# Autodesk Inventor assembly: MOTOR ENSAMBLE
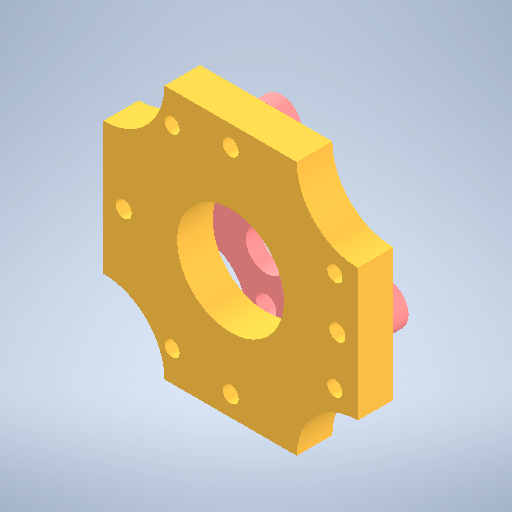
[picture p0: Inventor's stored thumbnail of the model, 512x512]
Saved by Autodesk Inventor 2025.3 (Build 293356030, 356C)
## iProperties
Created: 2025-07-11
Part Number: MOTOR ENSAMBLE
Document SubType Name: Assembly
Designer: jv
Author: jv
## Documents named in this file (3)
- C:\Users\jv\Downloads\MODELOS NUEVOS\MOTOR\MOTOR ENSAMBLE.iam
- C:\Users\jv\Downloads\MODELOS NUEVOS\MOTOR\CONECTOR DE ACOPLE A AVION.ipt
- C:\Users\jv\Downloads\MODELOS NUEVOS\MOTOR\ACOPLE.ipt
## Components (2 placed, 2 different names)
1. CONECTOR DE ACOPLE A AVION:1 — Mate:1
2. ACOPLE:1 — Mate:1
## Relationships (1: Mate 1)
- Mate:1: CONECTOR DE ACOPLE A AVION:1 ↔ ACOPLE:1
